# Autodesk Inventor assembly: sled plexi
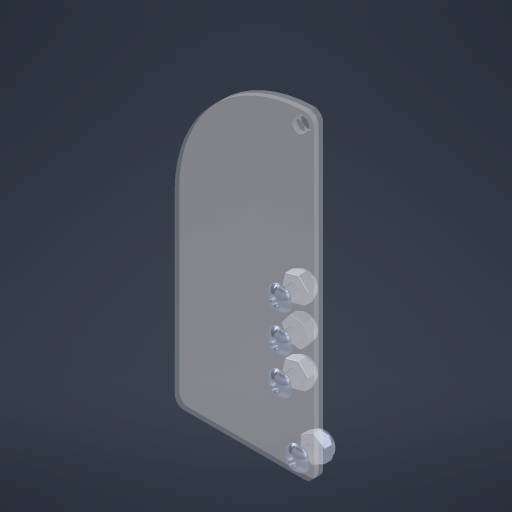
[picture p0: Inventor's stored thumbnail of the model, 512x512]
Saved by Autodesk Inventor 2023 (Build 270158000, 158)
## iProperties
Created: 2023-08-07
Part Number: sled plexi
Document SubType Name: Assembly
Designer: srbel
Author: srbel
## Documents named in this file (5)
- C:\CAD\OverUnderCAD\Drive\sled plexi.iam
- C:\CAD Robotics Season 23-24\sleds.ipt
- C:\CAD\OverUnderCAD\VEX-CAD-Inventor-1.4.0\Structure\Hardware\Screw Steel - Star\SScrew Star Threaded .290.ipt
- C:\CAD\OverUnderCAD\VEX-CAD-Inventor-1.4.0\Structure\Hardware\Screw Steel - Star.ipt
- C:\CAD\OverUnderCAD\VEX-CAD-Inventor-1.4.0\Structure\Hardware\Nut Thin Nylock.ipt
## Components (10 placed, 3 different names)
1. sleds:1 — Insert:1, Insert:2, Insert:7, Insert:8, Insert:9, Insert:10
2. sleds:2 — Insert:1, Insert:2, Insert:3, Insert:4, Insert:5, Insert:6
3. SScrew Star Threaded .290:1 — Insert:4
4. SScrew Star Threaded .290:2 — Insert:3
5. SScrew Star Threaded .290:3 — Insert:6
6. SScrew Star Threaded .290:4 — Insert:5
7. Nut Thin Nylock:1 — Insert:10
8. Nut Thin Nylock:2 — Insert:7
9. Nut Thin Nylock:3 — Insert:8
10. Nut Thin Nylock:4 — Insert:9
## Relationships (10: Insert 10)
- Insert:1: sleds:1 ↔ sleds:2
- Insert:2: sleds:1 ↔ sleds:2
- Insert:3: sleds:2 ↔ SScrew Star Threaded .290:2
- Insert:4: sleds:2 ↔ SScrew Star Threaded .290:1
- Insert:5: sleds:2 ↔ SScrew Star Threaded .290:4
- Insert:6: sleds:2 ↔ SScrew Star Threaded .290:3
- Insert:7 (1.5875 mm): sleds:1 ↔ Nut Thin Nylock:2
- Insert:8 (1.5875 mm): sleds:1 ↔ Nut Thin Nylock:3
- Insert:9 (1.5875 mm): sleds:1 ↔ Nut Thin Nylock:4
- Insert:10 (1.5875 mm): sleds:1 ↔ Nut Thin Nylock:1
